# Autodesk Inventor assembly: Assembly 8_14 finger
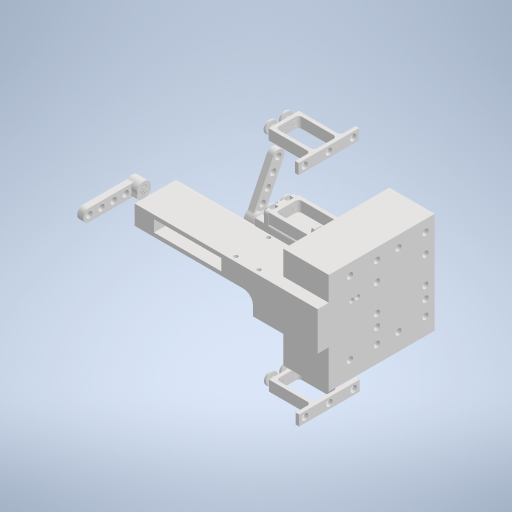
[picture p0: Inventor's stored thumbnail of the model, 512x512]
Saved by Autodesk Inventor 2024.2 (Build 282272000, 272)
## iProperties
Created: 2024-08-14
Part Number: Assembly 8_14 finger
Document SubType Name: Assembly
Designer: Tom
Author: Tom
## Documents named in this file (5)
- C:\Users\Tom\Desktop\UCSF\Preeya UCB\stretchable project\bender\Assembly 8_14 finger.iam
- C:\Users\Tom\Desktop\UCSF\Preeya UCB\stretchable project\bender\mcp pip plate.ipt
- C:\Users\Tom\Desktop\UCSF\Preeya UCB\stretchable project\bender\bender v2\servo_horz_mount\servo_horz_mount.ipt
- C:\Users\Tom\Desktop\UCSF\Preeya UCB\stretchable project\bender\bender v2\servo bilda\servo bilda.ipt
- C:\Users\Tom\Desktop\UCSF\Preeya UCB\stretchable project\bender\servo_arm\servo_arm.ipt
## Components (6 placed, 4 different names)
1. mcp pip plate:1 — Mate:1, Angle:1, Angle:2, Cylindrical:1, Angle:4, Insert:3
2. servo_horz_mount:1 — Mate:1, Angle:1, Cylindrical:1, Angle:3
3. servo_horz_mount:2 — Angle:2, Insert:2, Insert:3
4. servo bilda:1 — Insert:2, Cylindrical:2, Angle:3, Mate:2
5. servo_arm:1 — Cylindrical:2, Mate:2
6. servo_arm:2 — Angle:4
## Relationships (10: Angle 4, Mate 2, Insert 2, CylindricalJoint 2)
- Mate:1: mcp pip plate:1 ↔ servo_horz_mount:1
- Angle:1 (0 deg): mcp pip plate:1 ↔ servo_horz_mount:1
- Angle:2 (180 deg): mcp pip plate:1 ↔ servo_horz_mount:2
- Insert:2: servo_horz_mount:2 ↔ servo bilda:1
- Cylindrical:1: mcp pip plate:1 ↔ servo_horz_mount:1
- Cylindrical:2: servo bilda:1 ↔ servo_arm:1
- Angle:3 (0 deg): servo_horz_mount:1 ↔ servo bilda:1
- Mate:2: servo bilda:1 ↔ servo_arm:1
- Angle:4 (180 deg): mcp pip plate:1 ↔ servo_arm:2
- Insert:3: mcp pip plate:1 ↔ servo_horz_mount:2
